# Autodesk Inventor assembly: Linear Slide Assembly 9in
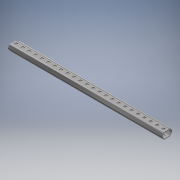
[picture p0: Inventor's stored thumbnail of the model, 180x180]
Saved by Autodesk Inventor 2017 (Build 210142000, 142)
## iProperties
Created: 2010-08-13
Part Number: Linear Slide Assembly 9in
Document SubType Name: Assembly
Designer: Hannah
Translation Standard: STEP AP203
FileName: Linear Slide Assembly.iam
PreProcessor: SolidWorks 2007
PostProcessor: Build: 239, Release: 2011 RTM - Date: Wed 02/17/2010
Sent Units: inch
Uncertainty: 1e-05
Author: Hannah
## Documents named in this file (3)
- E:\New Laptop\(1) New Laptop\AFNAN ALI flashdrive backup\VEXPARTS\Vex parts\Metal Other\Linear Slide Assembly 9in.iam
- E:\New Laptop\(1) New Laptop\AFNAN ALI flashdrive backup\VEXPARTS\Vex parts\Metal Other\Linear Slide Assembly-Parts\Linear Slide-Inner.ipt
- E:\New Laptop\(1) New Laptop\AFNAN ALI flashdrive backup\VEXPARTS\Vex parts\Metal Other\Linear Slide Assembly-Parts\Linear Slide-Outer.ipt
## Components (2 placed, 2 different names)
1. Linear Slide-Outer:1 — Mate:1, Flush:1
2. Linear Slide-Inner:1 — Mate:1, Flush:1
## Relationships (2: Mate 1, Flush 1)
- Mate:1 (10.16 mm): Linear Slide-Outer:1 ↔ Linear Slide-Inner:1
- Flush:1: Linear Slide-Outer:1 ↔ Linear Slide-Inner:1
